# Autodesk Inventor assembly: BotMockup
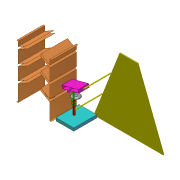
[picture p0: Inventor's stored thumbnail of the model, 180x180]
Saved by Autodesk Inventor 2012 (Build 160160000, 160)
## iProperties
Created: 2013-01-12
Part Number: BotMockup
Document SubType Name: Assembly
Designer: JesseK
Author: JesseK
## Documents named in this file (8)
- Z:\UserData\Documents\Inventor\team1885frc\Robot2013\sketches\BotMockup.iam
- Z:\UserData\Documents\Inventor\team1885frc\Robot2013\sketches\BaseMockup.ipt
- Z:\UserData\Documents\Inventor\team1885frc\Robot2013\sketches\VerticalTower.ipt
- Z:\UserData\Documents\Inventor\team1885frc\Robot2013\sketches\InnerTelescopeMockup.ipt
- Z:\UserData\Documents\Inventor\team1885frc\Robot2013\sketches\PyramidMockup.ipt
- Z:\UserData\Documents\Inventor\team1885frc\Robot2013\sketches\LauncherMockup.ipt
- Z:\UserData\Documents\Inventor\team1885frc\Robot2013\sketches\FeederMockup.ipt
- Z:\UserData\Documents\Inventor\team1885frc\Robot2013\Game\disc.ipt
## Components (10 placed, 7 different names)
1. BaseMockup:1 — Mate:1, Flush:1, Flush:2, Mate:10, Mate:11, Flush:5
2. VerticalTower:1 — Mate:1, Flush:1, Flush:2, Mate:8, Mate:9, Mate:12
3. InnerTelescopeMockup:1 — Mate:5, Flush:4, Mate:8, Mate:9, Mate:11, Mate:12
4. PyramidMockup:1 — Mate:10, Flush:6
5. LauncherMockup:1 — Mate:5, Flush:4
6. FeederMockup:1 — Flush:5, Flush:6, Flush:7, Flush:8, Flush:9
7. FeederMockup:2 — Flush:7, Flush:8
8. disc:1
9. disc:2 — Flush:9
10. disc:3
## Relationships (15: Flush 8, Mate 7)
- Mate:1: BaseMockup:1 ↔ VerticalTower:1
- Flush:1 (355.6 mm): BaseMockup:1 ↔ VerticalTower:1
- Flush:2 (368.3 mm): BaseMockup:1 ↔ VerticalTower:1
- Mate:5: InnerTelescopeMockup:1 ↔ LauncherMockup:1
- Flush:4 (-101.6 mm): InnerTelescopeMockup:1 ↔ LauncherMockup:1
- Mate:8: VerticalTower:1 ↔ InnerTelescopeMockup:1
- Mate:9: VerticalTower:1 ↔ InnerTelescopeMockup:1
- Mate:10: BaseMockup:1 ↔ PyramidMockup:1
- Mate:11 (50.8 mm): BaseMockup:1 ↔ InnerTelescopeMockup:1
- Flush:5: BaseMockup:1 ↔ FeederMockup:1
- Flush:6: PyramidMockup:1 ↔ FeederMockup:1
- Flush:7: FeederMockup:1 ↔ FeederMockup:2
- Flush:8: FeederMockup:1 ↔ FeederMockup:2
- Flush:9: FeederMockup:1 ↔ disc:2
- Mate:12: VerticalTower:1 ↔ InnerTelescopeMockup:1
